# Autodesk Inventor assembly: Assembly2
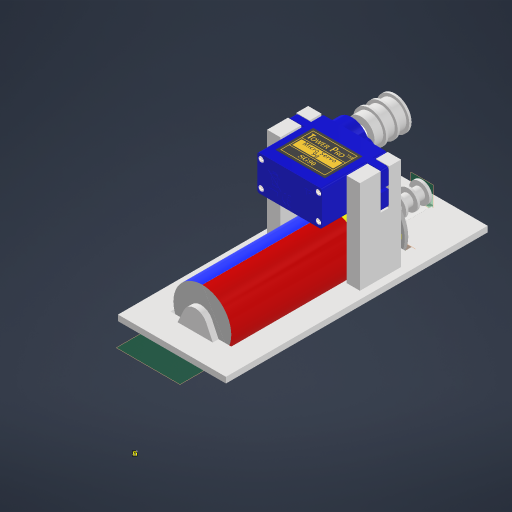
[picture p0: Inventor's stored thumbnail of the model, 512x512]
Saved by Autodesk Inventor 2024.3 (Build 283343000, 343)
## iProperties
Created: 2025-08-18
Part Number: Assembly2
Document SubType Name: Assembly
Designer: giuseppe
Author: giuseppe
## Documents named in this file (6)
- C:\Users\giuseppe\Desktop\Buckshot-Ruolette\CAD\mostra cartucce\V2\Assembly2.iam
- C:\Users\giuseppe\Desktop\Buckshot-Ruolette\CAD\mostra cartucce\rotater shell v3.ipt
- C:\Users\giuseppe\Desktop\Buckshot-Ruolette\CAD\mostra cartucce\V2\holderV2.ipt
- C:\Users\giuseppe\Desktop\Buckshot-Ruolette\CAD\mostra cartucce\V2\puleggia.ipt
- C:\Users\giuseppe\Desktop\Buckshot-Ruolette\CAD\mostra cartucce\SG90 - Micro Servo 9g - Tower Pro.1\SG90 - Micro Servo 9g - Tower Pro.1\SG90 - Micro Servo 9g - Tower Pro.1.ipt
- C:\Users\giuseppe\Desktop\Buckshot-Ruolette\CAD\mostra cartucce\V2\puleggia motore.ipt
## Components (5 placed, 5 different names)
1. rotater shell v3:1 — Flush:1, Flush:2, Flush:3, Flush:5
2. holderV2:1 — Flush:1, Flush:2, Flush:4, Mate:1, Flush:6, Mate:2, Flush:7, Flush:8
3. puleggia:1 — Flush:3, Flush:4, Flush:6, Flush:8
4. SG90 - Micro Servo 9g - Tower Pro.1:1 — Mate:1, Flush:5, Mate:2, Flush:7, Flush:9
5. puleggia motore:1 — Flush:9
## Relationships (11: Flush 9, Mate 2)
- Flush:1: rotater shell v3:1 ↔ holderV2:1
- Flush:2: rotater shell v3:1 ↔ holderV2:1
- Flush:3: rotater shell v3:1 ↔ puleggia:1
- Flush:4: holderV2:1 ↔ puleggia:1
- Mate:1 (30 mm): holderV2:1 ↔ SG90 - Micro Servo 9g - Tower Pro.1:1
- Flush:5: rotater shell v3:1 ↔ SG90 - Micro Servo 9g - Tower Pro.1:1
- Flush:6: holderV2:1 ↔ puleggia:1
- Mate:2 (20 mm): holderV2:1 ↔ SG90 - Micro Servo 9g - Tower Pro.1:1
- Flush:7 (2.61 mm): holderV2:1 ↔ SG90 - Micro Servo 9g - Tower Pro.1:1
- Flush:8 (0.5 mm): holderV2:1 ↔ puleggia:1
- Flush:9: SG90 - Micro Servo 9g - Tower Pro.1:1 ↔ puleggia motore:1
